# Autodesk Inventor assembly: YZ_Roller_Assemblie
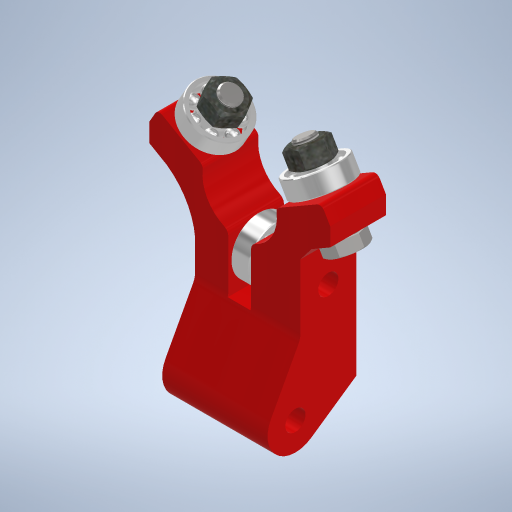
[picture p0: Inventor's stored thumbnail of the model, 512x512]
Saved by Autodesk Inventor 2023 (Build 270158000, 158)
## iProperties
Created: 2023-11-24
Part Number: YZ_Roller_Assemblie
Document SubType Name: Assembly
Designer: danie
Author: danie
## Documents named in this file (5)
- D:\Diplomarbeit\3d-model\basis_roboter\low_rider_v2\custom_files\YZ_Roller_Assemblie.iam
- D:\Diplomarbeit\3d-model\Imported Components\YZ_Roller\YZ_Roller.ipt
- D:\Diplomarbeit\3d-model\basis_roboter\low_rider_v2\custom_files\Bearing.ipt
- C:\Users\danie\OneDrive\Documents\Inventor\Content Center Files\R2023\en-US\ISO 8676(2)\ISO 8676 - M8 x 1 x 30 - ISO.ipt
- C:\Users\danie\OneDrive\Documents\Inventor\Content Center Files\R2023\en-US\ISO 8674(2)\ISO 8674 - M8 x 1ISO.ipt
## Components (8 placed, 4 different names)
1. YZ_Roller:1 — Rigid:1, Rigid:2, Rigid:3, Mate:1, Mate:2, Mate:3, Mate:5, Mate:6, Mate:7
2. Bearing:1 — Rigid:1, Mate:8
3. Bearing:2 — Rigid:2
4. Bearing:3 — Rigid:3, Mate:4
5. ISO 8676 M8 x 1 x 30:1 — Mate:1, Mate:2
6. ISO 8674 M8 x 1:1 — Mate:3, Mate:4
7. ISO 8676 M8 x 1 x 30:2 — Mate:5, Mate:6
8. ISO 8674 M8 x 1:2 — Mate:7, Mate:8
## Relationships (11: Mate 8, WeldJoint 3)
- Rigid:1 [WeldJoint]: YZ_Roller:1 ↔ Bearing:1
- Rigid:2 [WeldJoint]: YZ_Roller:1 ↔ Bearing:2
- Rigid:3 [WeldJoint]: YZ_Roller:1 ↔ Bearing:3
- Mate:1: YZ_Roller:1 ↔ ISO 8676 M8 x 1 x 30:1
- Mate:2: YZ_Roller:1 ↔ ISO 8676 M8 x 1 x 30:1
- Mate:3: YZ_Roller:1 ↔ ISO 8674 M8 x 1:1
- Mate:4: Bearing:3 ↔ ISO 8674 M8 x 1:1
- Mate:5: YZ_Roller:1 ↔ ISO 8676 M8 x 1 x 30:2
- Mate:6: YZ_Roller:1 ↔ ISO 8676 M8 x 1 x 30:2
- Mate:7: YZ_Roller:1 ↔ ISO 8674 M8 x 1:2
- Mate:8: Bearing:1 ↔ ISO 8674 M8 x 1:2
